# Autodesk Inventor assembly: esp+pines
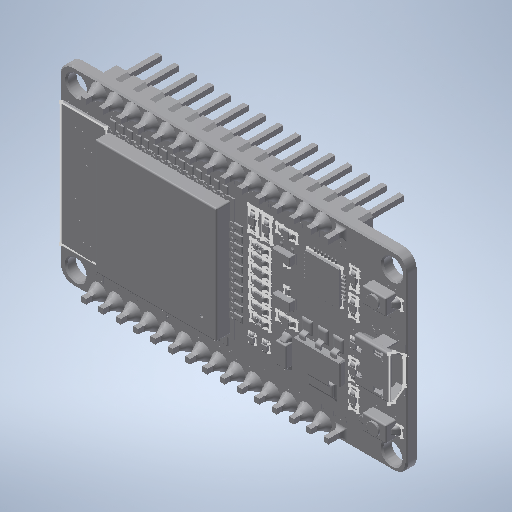
[picture p0: Inventor's stored thumbnail of the model, 512x512]
Saved by Autodesk Inventor 2025.2 (Build 292293000, 293)
## iProperties
Created: 2025-10-17
Part Number: esp+pines
Material: Generic
Document SubType Name: Assembly
Designer: Ricardo
Author: Ricardo
## Documents named in this file (3)
- C:\Users\Ricardo\Documents\Inventor\TFC\Componentes\female-pin-header-1.snapshot.1\2-Pin Header - Female - 2.54mm\2-Pin Header - Female - 2.54mm\esp+pines.iam
- C:\Users\Ricardo\Documents\Inventor\TFC\Componentes\esp32_devkitv1-1.snapshot.7\ESP32_DevKitV1\ESP32_en.ipt
- C:\Users\Ricardo\Documents\Inventor\TFC\Componentes\female-pin-header-1.snapshot.1\2pin_en.iam
## Components (2 placed, 2 different names)
1. ESP32_en:1 — Flush:1, Mate:1
2. 2pin_en:1 [sub-assembly] — Flush:1, Mate:1
## Relationships (2: Flush 1, Mate 1)
- Flush:1: ESP32_en:1 ↔ 2pin_en:1
- Mate:1: ESP32_en:1 ↔ 2pin_en:1
